# Autodesk Inventor assembly: CompleteSystem
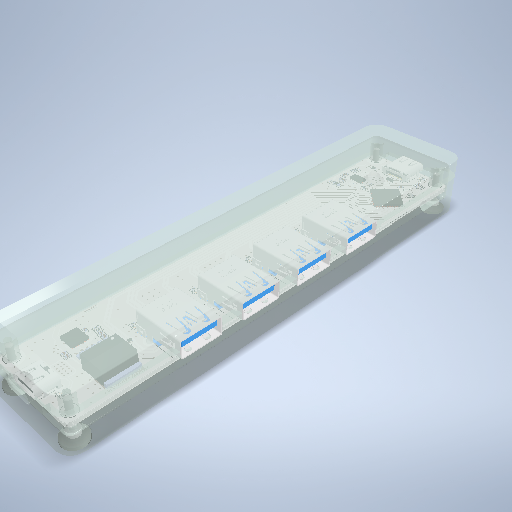
[picture p0: Inventor's stored thumbnail of the model, 512x512]
Saved by Autodesk Inventor 2025.1 (Build 291241020, 241B)
## iProperties
Created: 2026-01-18
Part Number: CompleteSystem
Document SubType Name: Assembly
Designer: JoaoVitorRamosMitidi
Author: JoaoVitorRamosMitidi
## Documents named in this file (6)
- C:\ProjectsOpenSource\USBHub3.2G1\Inventor_Project\CompleteSystem_ForBlender.iam
- C:\ProjectsOpenSource\USBHub3.2G1\Inventor_Project\Structure\Lower_Housing.ipt
- C:\ProjectsOpenSource\USBHub3.2G1\Inventor_Project\Structure\Upper_Housing.ipt
- C:\ProjectsOpenSource\USBHub3.2G1\Inventor_Project\Components\Rubber_Feet.ipt
- C:\ProjectsOpenSource\USBHub3.2G1\Inventor_Project\Components\DIN 7985 (H) - M2x10-H.ipt
- C:\ProjectsOpenSource\USBHub3.2G1\Inventor_Project\Board\USBHub3.2G1_ForBlender.ipt
## Components (12 placed, 5 different names)
1. USBHub3.2G1_ForBlender:1 — Alinhado:1, Inserir:12, Inserir:13
2. Lower_Housing:1 — Inserir:3, Inserir:4, Inserir:5, Inserir:6, Inserir:7, Inserir:8, Inserir:9, Inserir:10, Inserir:11, Alinhado:1, Inserir:12, Inserir:13
3. Upper_Housing:1
4. DIN 7985 (H) M2x10-H:5 — Inserir:3
5. DIN 7985 (H) M2x10-H:6 — Inserir:4
6. DIN 7985 (H) M2x10-H:7 — Inserir:5
7. DIN 7985 (H) M2x10-H:8 — Inserir:6
8. Rubber_Feet:1 — Inserir:10
9. Rubber_Feet:2 — Inserir:9
10. Rubber_Feet:3 — Inserir:8
11. Rubber_Feet:4 — Inserir:7
12. Rubber_Feet:5 — Inserir:11
## Relationships (12: Insert 11, Flush 1)
- Inserir:3: Lower_Housing:1 ↔ DIN 7985 (H) M2x10-H:5
- Inserir:4: Lower_Housing:1 ↔ DIN 7985 (H) M2x10-H:6
- Inserir:5: Lower_Housing:1 ↔ DIN 7985 (H) M2x10-H:7
- Inserir:6: Lower_Housing:1 ↔ DIN 7985 (H) M2x10-H:8
- Inserir:7: Lower_Housing:1 ↔ Rubber_Feet:4
- Inserir:8: Lower_Housing:1 ↔ Rubber_Feet:3
- Inserir:9: Lower_Housing:1 ↔ Rubber_Feet:2
- Inserir:10: Lower_Housing:1 ↔ Rubber_Feet:1
- Inserir:11: Lower_Housing:1 ↔ Rubber_Feet:5
- Alinhado:1 [Flush]: USBHub3.2G1_ForBlender:1 ↔ Lower_Housing:1
- Inserir:12: USBHub3.2G1_ForBlender:1 ↔ Lower_Housing:1
- Inserir:13: USBHub3.2G1_ForBlender:1 ↔ Lower_Housing:1
